# Autodesk Inventor assembly: 2014 Recycle Rush Robot 1
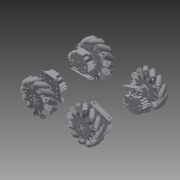
[picture p0: Inventor's stored thumbnail of the model, 180x180]
Saved by Autodesk Inventor 2014 (Build 180170000, 170)
## iProperties
Created: 2015-01-09
Part Number: 2014 Recycle Rush Robot 1
Document SubType Name: Assembly
Designer: student
Author: student
## Documents named in this file (9)
- C:\Users\student\Documents\Inventor\2015 Recycle Rush\2014 Recycle Rush Robot.iam
- C:\Users\student\Documents\Inventor\Dillon And Justin\Imported Components\am-0077a-500 Key Hub r2\am-0077a-500 Key Hub r2.ipt
- C:\Users\student\Documents\Inventor\Dillon And Justin\Imported Components\Toughbox mini (am-0654)\Toughbox mini (am-0654).iam
- C:\Users\student\Documents\Inventor\Dillon And Justin\Imported Components\8 inch mecanum left wheel\8 inch mecanum left wheel.iam
- C:\Users\student\Documents\Inventor\Dillon And Justin\Imported Components\8 inch mecanum right wheel\8 inch mecanum right wheel.iam
- C:\Users\student\Documents\Inventor\Dillon And Justin\Imported Components\am-0077a-500 Key Hub r2\am-0077a-500 Key Hub r2_MIR.ipt
- C:\Users\student\Documents\Inventor\Dillon And Justin\Imported Components\Toughbox mini (am-0654)\Toughbox mini (am-0654)_MIR.iam
- C:\Users\student\Documents\Inventor\Dillon And Justin\Imported Components\8 inch mecanum left wheel\8 inch mecanum left wheel_MIR.iam
- C:\Users\student\Documents\Inventor\Dillon And Justin\Imported Components\8 inch mecanum right wheel\8 inch mecanum right wheel_MIR.iam
## Components (12 placed, 8 different names)
1. 8 inch mecanum right wheel:1 [sub-assembly] — Mate:9, Mate:10, Mate:16
2. am-0077a-500 Key Hub r2:2 — Mate:9, Mate:10, Mate:11, Mate:12, Mate:16
3. Toughbox mini (am-0654):2 [sub-assembly] — Mate:11, Mate:12
4. 8 inch mecanum left wheel:2 [sub-assembly] — Mate:13, Mate:14
5. am-0077a-500 Key Hub r2:3 — Mate:13, Mate:14, Mate:15
6. Toughbox mini (am-0654):3 [sub-assembly] — Mate:15
7. am-0077a-500 Key Hub r2_MIR:1 — Mate:21, Mate:22, Mate:23, Mate:24, Mate:25
8. Toughbox mini (am-0654)_MIR:1 [sub-assembly] — Mate:21, Mate:22
9. 8 inch mecanum left wheel_MIR:1 [sub-assembly] — Mate:23, Mate:24, Mate:25
10. 8 inch mecanum right wheel_MIR:1 [sub-assembly] — Mate:26, Mate:27, Mate:28
11. am-0077a-500 Key Hub r2_MIR:2 — Mate:26, Mate:27, Mate:28, Mate:29
12. Toughbox mini (am-0654)_MIR:2 [sub-assembly] — Mate:29
## Relationships (17: Mate 17)
- Mate:9: 8 inch mecanum right wheel:1 ↔ am-0077a-500 Key Hub r2:2
- Mate:10: 8 inch mecanum right wheel:1 ↔ am-0077a-500 Key Hub r2:2
- Mate:11: am-0077a-500 Key Hub r2:2 ↔ Toughbox mini (am-0654):2
- Mate:12: am-0077a-500 Key Hub r2:2 ↔ Toughbox mini (am-0654):2
- Mate:13: 8 inch mecanum left wheel:2 ↔ am-0077a-500 Key Hub r2:3
- Mate:14: 8 inch mecanum left wheel:2 ↔ am-0077a-500 Key Hub r2:3
- Mate:15: am-0077a-500 Key Hub r2:3 ↔ Toughbox mini (am-0654):3
- Mate:16: 8 inch mecanum right wheel:1 ↔ am-0077a-500 Key Hub r2:2
- Mate:21: am-0077a-500 Key Hub r2_MIR:1 ↔ Toughbox mini (am-0654)_MIR:1
- Mate:22: am-0077a-500 Key Hub r2_MIR:1 ↔ Toughbox mini (am-0654)_MIR:1
- Mate:23: am-0077a-500 Key Hub r2_MIR:1 ↔ 8 inch mecanum left wheel_MIR:1
- Mate:24: am-0077a-500 Key Hub r2_MIR:1 ↔ 8 inch mecanum left wheel_MIR:1
- Mate:25: am-0077a-500 Key Hub r2_MIR:1 ↔ 8 inch mecanum left wheel_MIR:1
- Mate:26: 8 inch mecanum right wheel_MIR:1 ↔ am-0077a-500 Key Hub r2_MIR:2
- Mate:27: 8 inch mecanum right wheel_MIR:1 ↔ am-0077a-500 Key Hub r2_MIR:2
- Mate:28: 8 inch mecanum right wheel_MIR:1 ↔ am-0077a-500 Key Hub r2_MIR:2
- Mate:29: am-0077a-500 Key Hub r2_MIR:2 ↔ Toughbox mini (am-0654)_MIR:2
